# Autodesk Inventor assembly: gasienica_zlozenie
(part 2 of 2)
- [Mate]: tuleja_TUF106040:70 ↔ M6_40_shaft:7
- [Flush] (7 mm): ramie_1_wahacza:7 ↔ M6_40_shaft:7
- [Mate]: tuleja_TUF106040:73 ↔ M6_40_shaft:8
- [Flush] (7 mm): ramie_2_wahacza:8 ↔ M6_40_shaft:8
- [Mate]: M6_nut_5mm:89 ↔ M6_40_shaft:7
- [Mate]: ramie_1_wahacza:7 ↔ M6_nut_5mm:89
- [Mate]: M6_40_shaft:7 ↔ M6_nut_5mm:90
- [Mate]: ramie_1_wahacza:8 ↔ M6_nut_5mm:90
- [Mate]: M6_40_shaft:8 ↔ M6_nut_5mm:91
- [Mate]: ramie_2_wahacza:7 ↔ M6_nut_5mm:91
- [Mate]: M6_40_shaft:8 ↔ M6_nut_5mm:92
- [Mate]: ramie_2_wahacza:8 ↔ M6_nut_5mm:92
- [Mate]: M6_40_shaft:7 ↔ tuleja_M6_M10_7:10
- [Mate]: M6_40_shaft:8 ↔ tuleja_M6_M10_7:11
- [Mate]: M6_1,25_pad:25 ↔ M6_1,25_pad:26
- [Mate]: M6_1,25_pad:25 ↔ M6_1,25_pad:26
- [Mate]: M6_40_shaft:7 ↔ M6_1,25_pad:25
- [Mate]: M6_1,25_pad:27 ↔ M6_1,25_pad:28
- [Mate]: M6_1,25_pad:27 ↔ M6_1,25_pad:28
- [Mate]: M6_40_shaft:7 ↔ M6_1,25_pad:27
- [Mate]: tuleja_TUF106040:70 ↔ M6_1,25_pad:27
- [Mate]: M6_1,25_pad:29 ↔ M6_1,25_pad:30
- [Mate]: M6_1,25_pad:29 ↔ M6_1,25_pad:30
- [Mate]: M6_40_shaft:8 ↔ M6_1,25_pad:29
- [Mate]: M6_1,25_pad:31 ↔ M6_1,25_pad:32
- [Mate]: M6_1,25_pad:31 ↔ M6_1,25_pad:32
- [Mate]: M6_40_shaft:8 ↔ M6_1,25_pad:31
- [Mate]: tuleja_TUF106040:73 ↔ M6_1,25_pad:31
- [Mate]: M5_70_shaft:10 ↔ M6_70_shaft:19
- [Flush]: M5_70_shaft:10 ↔ M6_70_shaft:20
- [Mate]: M6_70_shaft:20 ↔ M6_nut_5mm:93
- [Mate]: M6_70_shaft:20 ↔ M6_nut_5mm:94
- [Mate] (60 mm): M6_nut_5mm:93 ↔ M6_nut_5mm:94
- [Flush]: M5_nut_5mm:64 ↔ M6_nut_5mm:94
- [Mate] (60 mm): M6_nut_5mm:95 ↔ M6_nut_5mm:96
- [Mate]: M6_nut_5mm:95 ↔ M6_nut_5mm:96
- [Mate]: M6_70_shaft:19 ↔ M6_nut_5mm:95
- [Flush]: M5_nut_5mm:64 ↔ M6_nut_5mm:96
- [Mate]: ramie_1_wahacza:7 ↔ M5_shaft:7
- [Flush] (7 mm): ramie_1_wahacza:7 ↔ M5_shaft:7
- [Mate]: ramie_1_wahacza:7 ↔ M5_shaft:8
- [Flush] (7 mm): ramie_1_wahacza:7 ↔ M5_shaft:8
- [Mate]: M5_shaft:8 ↔ M5_nut_5mm:66
- [Mate]: ramie_1_wahacza:7 ↔ M5_nut_5mm:66
- [Mate]: M5_shaft:7 ↔ M5_nut_5mm:67
- [Mate]: ramie_1_wahacza:7 ↔ M5_nut_5mm:67
- [Mate]: M5_shaft:7 ↔ M5_nut_5mm:68
- [Mate]: ramie_1_wahacza:8 ↔ M5_nut_5mm:68
- [Mate]: M5_shaft:8 ↔ M5_nut_5mm:69
- [Mate]: ramie_1_wahacza:8 ↔ M5_nut_5mm:69
- [Mate]: M5_shaft:7 ↔ tuleja_M5_M9_4,5:13
- [Mate]: ramie_1_wahacza:8 ↔ tuleja_M5_M9_4,5:13
- [Mate]: M5_shaft:7 ↔ tuleja_M5_M9_4,5:14
- [Mate]: ramie_1_wahacza:7 ↔ tuleja_M5_M9_4,5:14
- [Mate]: M5_shaft:8 ↔ tuleja_M5_M9_4,5:15
- [Mate]: ramie_1_wahacza:8 ↔ tuleja_M5_M9_4,5:15
- [Mate]: M5_shaft:8 ↔ tuleja_M5_M9_4,5:16
- [Mate]: ramie_1_wahacza:7 ↔ tuleja_M5_M9_4,5:16
- [Mate]: M6_40_shaft:8 ↔ glowny_wahacz_zewn:7
- [Mate]: tuleja_M6_M10_7:11 ↔ glowny_wahacz_zewn:7
- [Mate]: M6_40_shaft:7 ↔ glowny_wahacz_zewn:7
- [Mate]: M6_40_shaft:8 ↔ glowny_wahacz_zewn:8
- [Mate]: M6_40_shaft:7 ↔ glowny_wahacz_zewn:8
- [Mate]: tuleja_TUF106040:72 ↔ M6_40_shaft:7
- [Mate]: M6_1,25_pad:28 ↔ glowny_wahacz_zewn:8
- [Mate]: M6_1,25_pad:32 ↔ glowny_wahacz_zewn:8
- [Mate]: tuleja_M6_M10_7:10 ↔ glowny_wahacz_zewn:7
- [Mate]: M6_1,25_pad:25 ↔ glowny_wahacz_zewn:7
- [Mate]: tuleja_TUF106040:72 ↔ M6_1,25_pad:26
- [Mate]: M6_1,25_pad:29 ↔ glowny_wahacz_zewn:7
- [Mate]: tuleja_TUF106040:67 ↔ M6_1,25_pad:30
- [Mate]: tuleja_TUF106040:71 ↔ ramie_1_wahacza:8
- [Mate]: tuleja_TUF106040:69 ↔ M6_70_shaft:20
- [Mate]: ramie_1_wahacza:7 ↔ tuleja_TUF106040:69
- [Mate]: ramie_1_wahacza:7 ↔ tuleja_TUF106040:69
- [Mate]: tuleja_TUF106040:68 ↔ M6_70_shaft:19
- [Mate]: ramie_2_wahacza:7 ↔ tuleja_TUF106040:68
- [Mate]: ramie_2_wahacza:7 ↔ tuleja_TUF106040:68
- [Mate]: tuleja_TUF106040:74 ↔ M6_70_shaft:19
- [Mate]: ramie_2_wahacza:8 ↔ tuleja_TUF106040:74
- [Mate]: ramie_2_wahacza:8 ↔ tuleja_TUF106040:74
- [Mate]: ramie_1_wahacza:8 ↔ M5_shaft:8
- [Mate]: M6_70_shaft:19 ↔ M6_nut_5mm:97
- [Mate] (5 mm): M6_nut_5mm:96 ↔ M6_nut_5mm:97
- [Mate]: M6_70_shaft:19 ↔ M6_nut_5mm:98
- [Mate] (5 mm): M6_nut_5mm:95 ↔ M6_nut_5mm:98
- [Mate]: M6_70_shaft:20 ↔ M6_nut_5mm:99
- [Mate] (5 mm): M6_nut_5mm:93 ↔ M6_nut_5mm:99
- [Mate]: M6_70_shaft:20 ↔ M6_nut_5mm:100
- [Mate] (5 mm): M6_nut_5mm:94 ↔ M6_nut_5mm:100
- [Mate]: M6_70_shaft:20 ↔ tuleja_M6_M10_6:13
- [Mate]: tuleja_M6_M10_6:13 ↔ M6_nut_5mm:99
- [Mate]: M6_70_shaft:19 ↔ tuleja_M6_M10_6:14
- [Mate]: tuleja_TUF106040:74 ↔ tuleja_M6_M10_6:14
- [Mate]: M6_70_shaft:19 ↔ tuleja_M6_M10_6:15
- [Mate]: tuleja_TUF106040:68 ↔ tuleja_M6_M10_6:15
- [Mate]: M6_70_shaft:20 ↔ tuleja_M6_M10_6:16
- [Mate]: tuleja_TUF106040:71 ↔ tuleja_M6_M10_6:16
- [Mate]: M5_70_shaft:10 ↔ M5_nut_5mm:70
- [Mate] (5 mm): M5_nut_5mm:64 ↔ M5_nut_5mm:70
- [Mate]: M5_70_shaft:10 ↔ M5_nut_5mm:71
- [Mate] (5 mm): M5_nut_5mm:65 ↔ M5_nut_5mm:71
- [Mate]: M5_70_shaft:10 ↔ tuleja_M5_M9_17.5:8
- [Mate]: M5_nut_5mm:71 ↔ tuleja_M5_M9_17.5:8
- [Mate]: M5_70_shaft:10 ↔ tuleja_M5_M9_17.5:7
- [Mate]: Korpus:10 ↔ tuleja_M5_M9_17.5:7
- Zestawiające:1632 [Mate]: plyta_boczna:1 ↔ M6_70_shaft:16
- Zestawiające:1633 [Mate]: plyta_boczna:1 ↔ M6_nut_5mm:75
- Zestawiające:1636 [Mate]: plyta_boczna:2 ↔ M6_70_shaft:15
- Zestawiające:1637 [Mate]: plyta_boczna:2 ↔ tuleja_M5_M9_17.5:3
- Kątowe:40 [Angle] (90 deg): ramie_1_wahacza:4 ↔ glowny_wahacz_zewn:3
- Zestawiające:1638 [Mate]: plyta_boczna:2 ↔ M5_nut_5mm:65
- Zestawiające:1639 [Mate]: plyta_boczna:2 ↔ M6_70_shaft:20
- Zestawiające:1640 [Mate]: plyta_boczna:2 ↔ M6_70_shaft:19
- Zestawiające:1641 [Mate]: plyta_boczna:2 ↔ tuleja_M5_M9_17.5:7
- Kątowe:41 [Angle] (90 deg): ramie_1_wahacza:7 ↔ glowny_wahacz_zewn:8
- [Mate]: ramie_2_wahacza:9 ↔ tuleja_TUF106040:75
- [Mate]: ramie_2_wahacza:9 ↔ tuleja_TUF106040:75
- [Angle] (0 deg): ramie_2_wahacza:9 ↔ tuleja_TUF106040:75
- [Mate]: ramie_1_wahacza:9 ↔ tuleja_TUF106040:78
- [Mate]: ramie_1_wahacza:9 ↔ tuleja_TUF106040:78
- [Angle] (0 deg): ramie_1_wahacza:9 ↔ tuleja_TUF106040:78
- [Mate]: ramie_2_wahacza:10 ↔ tuleja_TUF106040:81
- [Mate]: ramie_2_wahacza:10 ↔ tuleja_TUF106040:81
- [Angle] (0 deg): ramie_2_wahacza:10 ↔ tuleja_TUF106040:81
- [Mate]: Korpus:11 ↔ Tlok:11
- [Angle] (0 deg): Korpus:11 ↔ Tlok:11
- [Mate]: Korpus:11 ↔ Nakretka:11
- [Mate] (5 mm): Korpus:11 ↔ Nakretka:11
- [CylindricalJoint]: Korpus:11 ↔ Tlok:11
- [Mate]: Korpus:11 ↔ M5_70_shaft:11
- [Flush] (-32.5 mm): Korpus:11 ↔ M5_70_shaft:11
- [Mate]: M5_nut_5mm:72 ↔ M5_70_shaft:11
- [Mate]: M5_70_shaft:11 ↔ M5_nut_5mm:73
- [Mate] (60 mm): M5_nut_5mm:72 ↔ M5_nut_5mm:73
- [Mate] (27.5 mm): Korpus:11 ↔ M5_nut_5mm:72
- [Mate]: tuleja_TUF106040:80 ↔ ramie_1_wahacza:10
- [Mate]: tuleja_TUF106040:79 ↔ ramie_1_wahacza:10
- [Mate]: tuleja_TUF106040:80 ↔ ramie_1_wahacza:10
- [Mate]: tuleja_TUF106040:75 ↔ tuleja_TUF106040:81
- [Mate]: wspornik_amortyzatora:21 ↔ wspornik_amortyzatora:22
- [Mate]: wspornik_amortyzatora:21 ↔ wspornik_amortyzatora:22
- [Mate] (5 mm): wspornik_amortyzatora:21 ↔ wspornik_amortyzatora:22
- [Mate]: M3_16_shaft:11 ↔ wspornik_amortyzatora:22
- [Flush] (-2.5 mm): M3_16_shaft:11 ↔ wspornik_amortyzatora:21
- [Mate]: M3_16_shaft:11 ↔ M3_nut_2,5mm:21
- [Mate]: M3_nut_2,5mm:21 ↔ wspornik_amortyzatora:21
- [Mate]: M3_16_shaft:11 ↔ M3_nut_2,5mm:22
- [Mate]: M3_nut_2,5mm:22 ↔ wspornik_amortyzatora:22
- [Mate]: Tlok:11 ↔ M3_16_shaft:11
- [Mate]: Tlok:11 ↔ wspornik_amortyzatora:22
- [Mate]: ramie_1_wahacza:9 ↔ wspornik_amortyzatora:21
- [Mate]: ramie_1_wahacza:9 ↔ wspornik_amortyzatora:21
- [Mate] (4.5 mm): ramie_1_wahacza:9 ↔ wspornik_amortyzatora:21
- [Mate]: tuleja_TUF106040:78 ↔ M6_40_shaft:9
- [Flush] (7 mm): ramie_1_wahacza:9 ↔ M6_40_shaft:9
- [Mate]: tuleja_TUF106040:81 ↔ M6_40_shaft:10
- [Flush] (7 mm): ramie_2_wahacza:10 ↔ M6_40_shaft:10
- [Mate]: M6_nut_5mm:101 ↔ M6_40_shaft:9
- [Mate]: ramie_1_wahacza:9 ↔ M6_nut_5mm:101
- [Mate]: M6_40_shaft:9 ↔ M6_nut_5mm:102
- [Mate]: ramie_1_wahacza:10 ↔ M6_nut_5mm:102
- [Mate]: M6_40_shaft:10 ↔ M6_nut_5mm:103
- [Mate]: ramie_2_wahacza:9 ↔ M6_nut_5mm:103
- [Mate]: M6_40_shaft:10 ↔ M6_nut_5mm:104
- [Mate]: ramie_2_wahacza:10 ↔ M6_nut_5mm:104
- [Mate]: M6_40_shaft:9 ↔ tuleja_M6_M10_7:13
- [Mate]: M6_40_shaft:10 ↔ tuleja_M6_M10_7:14
- [Mate]: M6_1,25_pad:33 ↔ M6_1,25_pad:34
- [Mate]: M6_1,25_pad:33 ↔ M6_1,25_pad:34
- [Mate]: M6_40_shaft:9 ↔ M6_1,25_pad:33
- [Mate]: M6_1,25_pad:35 ↔ M6_1,25_pad:36
- [Mate]: M6_1,25_pad:35 ↔ M6_1,25_pad:36
- [Mate]: M6_40_shaft:9 ↔ M6_1,25_pad:35
- [Mate]: tuleja_TUF106040:78 ↔ M6_1,25_pad:35
- [Mate]: M6_1,25_pad:37 ↔ M6_1,25_pad:38
- [Mate]: M6_1,25_pad:37 ↔ M6_1,25_pad:38
- [Mate]: M6_40_shaft:10 ↔ M6_1,25_pad:37
- [Mate]: M6_1,25_pad:39 ↔ M6_1,25_pad:40
- [Mate]: M6_1,25_pad:39 ↔ M6_1,25_pad:40
- [Mate]: M6_40_shaft:10 ↔ M6_1,25_pad:39
- [Mate]: tuleja_TUF106040:81 ↔ M6_1,25_pad:39
- [Mate]: M5_70_shaft:11 ↔ M6_70_shaft:21
- [Flush]: M5_70_shaft:11 ↔ M6_70_shaft:22
- [Mate]: M6_70_shaft:22 ↔ M6_nut_5mm:105
- [Mate]: M6_70_shaft:22 ↔ M6_nut_5mm:106
- [Mate] (60 mm): M6_nut_5mm:105 ↔ M6_nut_5mm:106
- [Flush]: M5_nut_5mm:72 ↔ M6_nut_5mm:106
- [Mate] (60 mm): M6_nut_5mm:107 ↔ M6_nut_5mm:108
- [Mate]: M6_nut_5mm:107 ↔ M6_nut_5mm:108
- [Mate]: M6_70_shaft:21 ↔ M6_nut_5mm:107
- [Flush]: M5_nut_5mm:72 ↔ M6_nut_5mm:108
- [Mate]: ramie_1_wahacza:9 ↔ M5_shaft:9
- [Flush] (7 mm): ramie_1_wahacza:9 ↔ M5_shaft:9
- [Mate]: ramie_1_wahacza:9 ↔ M5_shaft:10
- [Flush] (7 mm): ramie_1_wahacza:9 ↔ M5_shaft:10
- [Mate]: M5_shaft:10 ↔ M5_nut_5mm:74
- [Mate]: ramie_1_wahacza:9 ↔ M5_nut_5mm:74
- [Mate]: M5_shaft:9 ↔ M5_nut_5mm:75
- [Mate]: ramie_1_wahacza:9 ↔ M5_nut_5mm:75
- [Mate]: M5_shaft:9 ↔ M5_nut_5mm:76
- [Mate]: ramie_1_wahacza:10 ↔ M5_nut_5mm:76
- [Mate]: M5_shaft:10 ↔ M5_nut_5mm:77
- [Mate]: ramie_1_wahacza:10 ↔ M5_nut_5mm:77
- [Mate]: M5_shaft:9 ↔ tuleja_M5_M9_4,5:17
- [Mate]: ramie_1_wahacza:10 ↔ tuleja_M5_M9_4,5:17
- [Mate]: M5_shaft:9 ↔ tuleja_M5_M9_4,5:18
- [Mate]: ramie_1_wahacza:9 ↔ tuleja_M5_M9_4,5:18
- [Mate]: M5_shaft:10 ↔ tuleja_M5_M9_4,5:19
- [Mate]: ramie_1_wahacza:10 ↔ tuleja_M5_M9_4,5:19
- [Mate]: M5_shaft:10 ↔ tuleja_M5_M9_4,5:20
- [Mate]: ramie_1_wahacza:9 ↔ tuleja_M5_M9_4,5:20
- [Mate]: M6_40_shaft:10 ↔ glowny_wahacz_zewn:9
- [Mate]: tuleja_M6_M10_7:14 ↔ glowny_wahacz_zewn:9
- [Mate]: M6_40_shaft:9 ↔ glowny_wahacz_zewn:9
- [Mate]: M6_40_shaft:10 ↔ glowny_wahacz_zewn:10
- [Mate]: M6_40_shaft:9 ↔ glowny_wahacz_zewn:10
- [Mate]: tuleja_TUF106040:80 ↔ M6_40_shaft:9
- [Mate]: M6_1,25_pad:36 ↔ glowny_wahacz_zewn:10
- [Mate]: M6_1,25_pad:40 ↔ glowny_wahacz_zewn:10
- [Mate]: tuleja_M6_M10_7:13 ↔ glowny_wahacz_zewn:9
- [Mate]: M6_1,25_pad:33 ↔ glowny_wahacz_zewn:9
- [Mate]: tuleja_TUF106040:80 ↔ M6_1,25_pad:34
- [Mate]: M6_1,25_pad:37 ↔ glowny_wahacz_zewn:9
- [Mate]: tuleja_TUF106040:75 ↔ M6_1,25_pad:38
- [Mate]: tuleja_TUF106040:79 ↔ ramie_1_wahacza:10
- [Mate]: tuleja_TUF106040:77 ↔ M6_70_shaft:22
- [Mate]: ramie_1_wahacza:9 ↔ tuleja_TUF106040:77
- [Mate]: ramie_1_wahacza:9 ↔ tuleja_TUF106040:77
- [Mate]: tuleja_TUF106040:76 ↔ M6_70_shaft:21
- [Mate]: ramie_2_wahacza:9 ↔ tuleja_TUF106040:76
- [Mate]: ramie_2_wahacza:9 ↔ tuleja_TUF106040:76
- [Mate]: tuleja_TUF106040:82 ↔ M6_70_shaft:21
- [Mate]: ramie_2_wahacza:10 ↔ tuleja_TUF106040:82
- [Mate]: ramie_2_wahacza:10 ↔ tuleja_TUF106040:82
- [Mate]: independent_wheel_pair:5 ↔ tuleja_M6_M10_7:15
- [Mate]: glowny_wahacz_zewn:10 ↔ independent_wheel_pair:5
- [Mate]: glowny_wahacz_zewn:10 ↔ independent_wheel_pair:5
- [Mate]: glowny_wahacz_zewn:10 ↔ tuleja_M6_M10_7:15
- [Mate]: ramie_1_wahacza:10 ↔ M5_shaft:10
- [Mate]: M6_70_shaft:21 ↔ M6_nut_5mm:109
- [Mate] (5 mm): M6_nut_5mm:108 ↔ M6_nut_5mm:109
- [Mate]: M6_70_shaft:21 ↔ M6_nut_5mm:110
- [Mate] (5 mm): M6_nut_5mm:107 ↔ M6_nut_5mm:110
- [Mate]: M6_70_shaft:22 ↔ M6_nut_5mm:111
- [Mate] (5 mm): M6_nut_5mm:105 ↔ M6_nut_5mm:111
- [Mate]: M6_70_shaft:22 ↔ M6_nut_5mm:112
- [Mate] (5 mm): M6_nut_5mm:106 ↔ M6_nut_5mm:112
- [Mate]: M6_70_shaft:22 ↔ tuleja_M6_M10_6:17
- [Mate]: tuleja_M6_M10_6:17 ↔ M6_nut_5mm:111
- [Mate]: M6_70_shaft:21 ↔ tuleja_M6_M10_6:18
- [Mate]: tuleja_TUF106040:82 ↔ tuleja_M6_M10_6:18
- [Mate]: M6_70_shaft:21 ↔ tuleja_M6_M10_6:19
- [Mate]: tuleja_TUF106040:76 ↔ tuleja_M6_M10_6:19
- [Mate]: M6_70_shaft:22 ↔ tuleja_M6_M10_6:20
- [Mate]: tuleja_TUF106040:79 ↔ tuleja_M6_M10_6:20
- [Mate]: M5_70_shaft:11 ↔ M5_nut_5mm:78
- [Mate] (5 mm): M5_nut_5mm:72 ↔ M5_nut_5mm:78
- [Mate]: M5_70_shaft:11 ↔ M5_nut_5mm:79
- [Mate] (5 mm): M5_nut_5mm:73 ↔ M5_nut_5mm:79
- [Mate]: M5_70_shaft:11 ↔ tuleja_M5_M9_17.5:10
- [Mate]: M5_nut_5mm:79 ↔ tuleja_M5_M9_17.5:10
- [Mate]: M5_70_shaft:11 ↔ tuleja_M5_M9_17.5:9
- [Mate]: Korpus:11 ↔ tuleja_M5_M9_17.5:9
- [Mate]: glowny_wahacz_zewn:9 ↔ independent_wheel_pair:5
- Zestawiające:1777 [Mate]: plyta_boczna:2 ↔ M6_nut_5mm:107
- Zestawiające:1778 [Mate]: plyta_boczna:2 ↔ M6_70_shaft:22
- Zestawiające:1779 [Mate]: plyta_boczna:2 ↔ M6_70_shaft:21
- Zestawiające:1780 [Mate]: plyta_boczna:2 ↔ tuleja_M5_M9_17.5:10
- Kątowe:47 [Angle] (90 deg): ramie_1_wahacza:9 ↔ glowny_wahacz_zewn:10
- Zestawiające:1781 [Mate]: glowny_wahacz_zewn:8 ↔ komplet_kol_V4:1
- Zestawiające:1782 [Mate]: glowny_wahacz_zewn:8 ↔ komplet_kol_V4:1
- Zestawiające:1784 [Mate]: glowny_wahacz_zewn:7 ↔ komplet_kol_V4:1
- [Mate]: M6_25_shaft:2 ↔ M6_nut_5mm:116
- [Mate]: M6_nut_5mm:115 ↔ M6_25_shaft:2
- [Flush] (-1 mm): M6_nut_5mm:115 ↔ M6_25_shaft:2
- [Flush] (1 mm): M6_25_shaft:2 ↔ M6_nut_5mm:116
- Zestawiające:1788 [Mate]: komplet_kol_V4:1 ↔ M6_25_shaft:2
- Zestawiające:1789 [Mate]: glowny_wahacz_zewn:8 ↔ M6_nut_5mm:115
- [Mate]: M6_25_shaft:3 ↔ M6_nut_5mm:118
- [Mate]: M6_nut_5mm:117 ↔ M6_25_shaft:3
- [Flush] (-1 mm): M6_nut_5mm:117 ↔ M6_25_shaft:3
- [Flush] (1 mm): M6_25_shaft:3 ↔ M6_nut_5mm:118
- [Mate]: komplet_kol_V4:2 ↔ M6_25_shaft:3
- Zestawiające:1793 [Mate] (7 mm): glowny_wahacz_zewn:3 ↔ glowny_wahacz_zewn:4
- Zestawiające:1794 [Mate]: glowny_wahacz_zewn:3 ↔ M6_25_shaft:3
- Zestawiające:1795 [Mate]: glowny_wahacz_zewn:3 ↔ komplet_kol_V4:2
- Kątowe:48 [Angle] (0 deg): komplet_kol_V4:1 ↔ komplet_kol_V4:2
- Kątowe:49 [Angle] (0 deg): plyta_boczna:1 ↔ komplet_kol_V4:2
- Zestawiające:1796 [Mate]: M5_60_shaft:2 ↔ tuleja_M5_M9_13:1
- Zestawiające:1797 [Mate]: M5_60_shaft:2 ↔ tuleja_M5_M9_18:1
- [Mate]: single_wheel_dummie:1 ↔ tuleja_M5_M10_15:1
- Zestawiające:1799 [Mate]: single_wheel_dummie:1 ↔ tuleja_M5_M10_15:1
- Zestawiające:1800 [Mate]: single_wheel_dummie:2 ↔ tuleja_M5_M10_15:1
- Zestawiające:1801 [Mate]: single_wheel_dummie:2 ↔ tuleja_M5_M10_15:1
- Zestawiające:1802 [Mate]: M6_70_shaft:11 ↔ single_wheel_dummie:2
- Zestawiające:1803 [Mate]: M6_70_shaft:11 ↔ tuleja_M6_M10_7,5:1
- Zestawiające:1804 [Mate]: ramie_napinacza:2 ↔ tuleja_M6_M10_7,5:1
- Zestawiające:1805 [Mate]: single_wheel_dummie:2 ↔ tuleja_M6_M10_7,5:1
- Zestawiające:1806 [Mate]: M6_70_shaft:11 ↔ tuleja_M6_M10_7,5:2
- Zestawiające:1807 [Mate]: ramie_napinacza:1 ↔ tuleja_M6_M10_7,5:2
## Named parameters: d25_d17_d47_d24 = 0 mm, d26_d18_d48_d25 = 0 mm, d27_d19_d15 = 0 mm, d28_d20_d16 = 5 mm, d102_d31 = 0 mm, d103_d32 = 7 mm, d104_d33 = 0 mm, d105_d34 = 0 mm, d705_d35 = 0 mm, d706_d36 = 31 mm, d707_d37 = 0 mm, d109_d23 = 0 mm, d110_d24 = 0 mm, d111_d25 = 0 mm, d112_d26 = 0 mm, d113_d27 = 7 mm, d114_d28 = 0 mm, d115_d30 = 0 mm, d715_d116 = 0 mm, d716_d117 = 0 mm, d717_d118 = 0 mm, d718_d119 = 0 mm, susp_angle = 90 deg, tlok_scisniety = -13 mm, tlok_wyprostowany = 1 mm, d1532_d239 = 0 mm, d1533_d174 = 0 mm, d1534_d175 = 0 mm, d1535_d176 = 60 mm, d1545_d86_d0 = 0 mm, d1546_d87_d1 = 0 deg, d1547_d88_d3 = 0 mm, d1548_d89_d4 = 5 mm, d1549_d90_d5 = 0 deg, d1550_d108 = 0 mm, d1551_d109 = -30 mm, d1552_d110 = 0 mm, d1553_d111 = 0 mm, d1554_d112 = 60 mm, d1555_d113 = 30 mm, d1587_d202 = 0 mm, d1588_d203 = 0 mm, d1589_d204 = 0 mm, d1590_d205 = 0 mm, d1591_d120 = 0 mm, d1592_d121 = 0 mm, d1593_d122 = 5 mm, d1594_d123 = 0 mm, d1595_d124 = -2.5 mm, d1596_d125 = 0 mm, d1597_d126 = 0 mm, d1598_d127 = 0 mm, d1599_d128 = 0 mm, d1600_d129 = 0 mm, d1601_d130 = 0 mm, d1602_d83_d6 = 0 mm, d1603_d84_d7 = -13 mm, d1604_d85_d8 = -13 mm, d1684_d208 = 0 mm, d1685_d209 = 0 mm, d158_d154 = 0 mm, d159_d155 = 0 mm, d162_d154 = 0 mm, d163_d155 = 0 mm, d166_d154 = 0 mm, d167_d155 = 0 mm, d178_d176 = 60 mm, d41_d4 = 0 deg, d43_d0 = 0 mm, d44_d1 = 0 mm, d83_d6 = 0 mm, d84_d7 = -5.94197 mm, d85_d8 = -13 mm, d86_d0 = 0 mm, d87_d1 = 0 deg, d88_d3 = 0 mm, d89_d4 = 5 mm, d90_d5 = 0 deg, d1784_d333 = 5 mm, d1785_d334 = 0 mm, d1786_d335 = 5 mm, d1787_d336 = 0 mm, d1788_d337 = 0 mm, d1789_d338 = 0 mm, d1790_d339 = 0 mm, d1792_d321 = 5 mm, d1793_d322 = 0 mm, d1794_d323 = 5 mm, d1795_d324 = 0 mm, d1796_d325 = 0 mm, d1797_d326 = 0 mm, d1798_d327 = 0 mm, d1799_d328 = 0 mm, d1800_d329 = 0 mm, d1801_d330 = 0 mm, d1802_d331 = 0 mm, d1803_d332 = 0 mm, d1804_d0 = 0 mm, d1805_d1 = 0 mm, d1806_d4 = 0 deg, d1807_d9 = 0 mm, d1808_d315 = 0 mm, d1809_d316 = 0 mm, d1810_d317 = 5 mm, d1811_d318 = 0 mm, d1812_d319 = 5 mm, d1813_d320 = 0 mm, d1814_d233 = 0 mm, d1815_d234 = 0 mm, d1816_d235 = 0 mm, d1817_d236 = 0 mm, d1818_d237 = 0 mm, d1819_d238 = 0 mm, d1820_d239 = 0 mm, d1821_d240 = 0 mm, d1822_d241 = 0 mm, d1823_d242 = 0 mm, d1824_d243 = 0 mm, d1825_d244 = 0 mm, d1826_d245 = 0 mm, d1827_d246 = 0 mm, d1828_d247 = 0 mm, d1833_d195 = 0 mm, d1834_d196 = 0 mm, d1835_d197 = 0 mm, d1836_d198 = 0 mm, d1837_d199 = 0 mm, d1838_d200 = 0 mm, d1839_d201 = 0 mm, d1840_d206 = 0 mm, d1841_d207 = 0 mm, d1842_d208 = 0 mm, d1843_d209 = 0 mm, d1844_d210 = 0 mm, d1845_d211 = 0 mm, d1846_d212 = 0 mm, d1847_d213 = 0 mm, d1848_d216 = 0 mm, d1849_d217 = 0 mm, d1850_d218 = 0 mm, d1851_d221 = 0 mm, d1852_d222 = 0 mm, d1853_d225 = 0 mm, d1854_d231 = 0 mm, d1855_d232 = 0 mm, d1856_d154 = 0 mm, d1857_d155 = 0 mm, d1858_d156 = 0 mm, d1859_d158_d154 = 0 mm, d1860_d159_d155 = 0 mm, d1861_d160 = 0 mm, d1862_d161 = 0 mm, d1863_d162_d154 = 0 mm, d1864_d163_d155 = 0 mm, d1865_d164 = 0 mm, d1866_d166_d154 = 0 mm, d1867_d167_d155 = 0 mm, d1868_d168 = 0 mm, d1869_d169 = 0 mm, d1870_d172 = 0 mm, d1871_d173 = 0 mm, d1872_d174 = 0 mm, d1873_d175 = 0 mm, d1874_d176 = 60 mm, d1875_d177 = 0 mm, d1876_d178_d176 = 60 mm, d1877_d179 = 0 mm, d1878_d180 = 0 mm, d1879_d181 = 0 mm, d1880_d190 = 0 mm, d1881_d191 = 7 mm, d1882_d192 = 0 mm, d1883_d193 = 7 mm, d1884_d194 = 0 mm, d1885_d119 = 0 mm, d1886_d120 = 0 mm, d1887_d121 = 0 mm, d1888_d122 = 5 mm, d1889_d123 = 0 mm, d1890_d124 = -2.5 mm, d1891_d125 = 0 mm, d1892_d126 = 0 mm, d1893_d127 = 0 mm, d1894_d128 = 0 mm, d1895_d129 = 0 mm, d1896_d130 = 0 mm, d1897_d135 = 0 mm, d1898_d136 = 0 mm, d1899_d137 = 4.5 mm, d1900_d138 = 0 mm, d1901_d139 = 7 mm, d1902_d140 = 0 mm, d1903_d141 = 7 mm, d1904_d142 = 0 mm, d1905_d143 = 0 mm, d1906_d144 = 0 mm, d1907_d145 = 0 mm, d1908_d146 = 0 mm, d1909_d147 = 0 mm, d1910_d148 = 0 mm, d1911_d149 = 0 mm, d1912_d150 = 0 mm, d1913_d152 = 0 mm, d1914_d10 = 0 mm, d1915_d11 = 0 deg, d1916_d41_d4 = 0 deg, d1917_d43_d0 = 0 mm, d1918_d44_d1 = 0 mm, d1919_d83_d6 = 0 mm, d1920_d84_d7 = -5.942 mm, d1921_d85_d8 = -13 mm, d1922_d86_d0 = 0 mm, d1923_d87_d1 = 0 deg, d1924_d88_d3 = 0 mm, d1925_d89_d4 = 5 mm, d1926_d90_d5 = 0 deg, d1927_d108 = 0 mm, d1928_d109 = -32.5 mm, d1929_d110 = 0 mm, d1930_d111 = 0 mm, d1931_d112 = 60 mm, d1932_d113 = 27.5 mm, d1933_d114 = 0 mm, d1934_d115 = 0 mm, d1935_d116 = 0 mm, d2088_d333 = 5 mm, d2089_d334 = 0 mm, d2090_d335 = 5 mm, d2091_d336 = 0 mm, d2092_d337 = 0 mm, d2093_d338 = 0 mm, d2094_d339 = 0 mm, d2096_d321 = 5 mm, d2097_d322 = 0 mm, d2098_d323 = 5 mm, d2099_d324 = 0 mm, d2100_d325 = 0 mm, d2101_d326 = 0 mm, d2102_d327 = 0 mm, d2103_d328 = 0 mm, d2104_d329 = 0 mm, d2105_d330 = 0 mm, d2106_d331 = 0 mm, d2107_d332 = 0 mm, d2108_d0 = 0 mm, d2109_d1 = 0 mm, d2110_d4 = 0 deg, d2111_d9 = 0 mm, d2112_d315 = 0 mm, d2113_d316 = 0 mm, d2114_d317 = 5 mm, d2115_d318 = 0 mm, d2116_d319 = 5 mm, d2117_d320 = 0 mm, d2118_d233 = 0 mm, d2119_d234 = 0 mm, d2120_d235 = 0 mm, d2121_d236 = 0 mm, d2122_d237 = 0 mm, d2123_d238 = 0 mm, d2124_d239 = 0 mm, d2125_d240 = 0 mm, d2126_d241 = 0 mm, d2127_d242 = 0 mm, d2128_d243 = 0 mm, d2129_d244 = 0 mm, d2130_d245 = 0 mm, d2131_d246 = 0 mm, d2132_d247 = 0 mm, d2137_d195 = 0 mm, d2138_d196 = 0 mm, d2139_d197 = 0 mm, d2140_d198 = 0 mm, d2141_d199 = 0 mm, d2142_d200 = 0 mm, d2143_d201 = 0 mm, d2144_d206 = 0 mm, d2145_d207 = 0 mm, d2146_d208 = 0 mm, d2147_d209 = 0 mm, d2148_d210 = 0 mm, d2149_d211 = 0 mm, d2150_d212 = 0 mm, d2151_d213 = 0 mm, d2152_d216 = 0 mm, d2153_d217 = 0 mm, d2154_d218 = 0 mm, d2155_d221 = 0 mm, d2156_d222 = 0 mm, d2157_d225 = 0 mm, d2158_d231 = 0 mm, d2159_d232 = 0 mm, d2160_d154 = 0 mm, d2161_d155 = 0 mm, d2162_d156 = 0 mm, d2163_d158_d154 = 0 mm, d2164_d159_d155 = 0 mm, d2165_d160 = 0 mm, d2166_d161 = 0 mm, d2167_d162_d154 = 0 mm, d2168_d163_d155 = 0 mm, d2169_d164 = 0 mm, d2170_d166_d154 = 0 mm, d2171_d167_d155 = 0 mm, d2172_d168 = 0 mm, d2173_d169 = 0 mm, d2174_d172 = 0 mm, d2175_d173 = 0 mm, d2176_d174 = 0 mm, d2177_d175 = 0 mm, d2178_d176 = 60 mm, d2179_d177 = 0 mm, d2180_d178_d176 = 60 mm, d2181_d179 = 0 mm, d2182_d180 = 0 mm, d2183_d181 = 0 mm, d2184_d190 = 0 mm, d2185_d191 = 7 mm, d2186_d192 = 0 mm, d2187_d193 = 7 mm, d2188_d194 = 0 mm, d2189_d119 = 0 mm, d2190_d120 = 0 mm, d2191_d121 = 0 mm, d2192_d122 = 5 mm, d2193_d123 = 0 mm, d2194_d124 = -2.5 mm, d2195_d125 = 0 mm, d2196_d126 = 0 mm, d2197_d127 = 0 mm, d2198_d128 = 0 mm, d2199_d129 = 0 mm, d2200_d130 = 0 mm, d2201_d135 = 0 mm, d2202_d136 = 0 mm, d2203_d137 = 4.5 mm, d2204_d138 = 0 mm, d2205_d139 = 7 mm, d2206_d140 = 0 mm, d2207_d141 = 7 mm, d2208_d142 = 0 mm, d2209_d143 = 0 mm, d2210_d144 = 0 mm, d2211_d145 = 0 mm, d2212_d146 = 0 mm, d2213_d147 = 0 mm, d2214_d148 = 0 mm, d2215_d149 = 0 mm, d2216_d150 = 0 mm, d2217_d152 = 0 mm, d2218_d10 = 0 mm, d2219_d11 = 0 deg, d2220_d41_d4 = 0 deg, d2221_d43_d0 = 0 mm, d2222_d44_d1 = 0 mm, d2223_d83_d6 = 0 mm, d2224_d84_d7 = -5.942 mm, d2225_d85_d8 = -13 mm, d2226_d86_d0 = 0 mm, d2227_d87_d1 = 0 deg, d2228_d88_d3 = 0 mm, d2229_d89_d4 = 5 mm, d2230_d90_d5 = 0 deg, d2231_d108 = 0 mm, d2232_d109 = -32.5 mm, d2233_d110 = 0 mm, d2234_d111 = 0 mm, d2235_d112 = 60 mm, d2236_d113 = 27.5 mm, d2237_d114 = 0 mm, d2238_d115 = 0 mm, d2239_d116 = 0 mm, d2252_d2088_d333 = 5 mm, d2253_d2089_d334 = 0 mm, d2254_d2090_d335 = 5 mm, d2255_d2091_d336 = 0 mm, d2256_d2092_d337 = 0 mm, d2257_d2093_d338 = 0 mm, d2258_d2094_d339 = 0 mm, d2259_d2095_d340 = 0 mm, d2260_d2096_d321 = 5 mm, d2261_d2097_d322 = 0 mm, d2262_d2098_d323 = 5 mm, d2263_d2099_d324 = 0 mm, d2264_d2100_d325 = 0 mm, d2265_d2101_d326 = 0 mm, d2266_d2102_d327 = 0 mm, d2267_d2103_d328 = 0 mm, d2268_d2104_d329 = 0 mm, d2269_d2105_d330 = 0 mm, d2270_d2106_d331 = 0 mm, d2271_d2107_d332 = 0 mm, d2272_d2108_d0 = 0 mm, d2273_d2109_d1 = 0 mm, d2274_d2110_d4 = 0 deg, d2275_d2111_d9 = 0 mm, d2276_d2112_d315 = 0 mm, d2277_d2113_d316 = 0 mm, d2278_d2114_d317 = 5 mm, d2279_d2115_d318 = 0 mm, d2280_d2116_d319 = 5 mm, d2281_d2117_d320 = 0 mm, d2282_d2118_d233 = 0 mm, d2283_d2119_d234 = 0 mm, d2284_d2120_d235 = 0 mm, d2285_d2121_d236 = 0 mm, d2286_d2122_d237 = 0 mm, d2287_d2123_d238 = 0 mm, d2288_d2124_d239 = 0 mm, d2289_d2125_d240 = 0 mm, d2290_d2126_d241 = 0 mm, d2291_d2127_d242 = 0 mm, d2292_d2128_d243 = 0 mm, d2293_d2129_d244 = 0 mm, d2294_d2130_d245 = 0 mm, d2295_d2131_d246 = 0 mm, d2296_d2132_d247 = 0 mm, d2297_d2133_d1369 = 0 mm, d2298_d2134_d260 = 0 mm, d2299_d2135_d261 = 0 mm, d2300_d2136_d262 = 0 mm, d2301_d2137_d195 = 0 mm, d2302_d2138_d196 = 0 mm, d2303_d2139_d197 = 0 mm, d2304_d2140_d198 = 0 mm, d2305_d2141_d199 = 0 mm, d2306_d2142_d200 = 0 mm, d2307_d2143_d201 = 0 mm, d2308_d2144_d206 = 0 mm, d2309_d2145_d207 = 0 mm, d2310_d2146_d208 = 0 mm, d2311_d2147_d209 = 0 mm, d2312_d2148_d210 = 0 mm, d2313_d2149_d211 = 0 mm, d2314_d2150_d212 = 0 mm, d2315_d2151_d213 = 0 mm, d2316_d2152_d216 = 0 mm, d2317_d2153_d217 = 0 mm, d2318_d2154_d218 = 0 mm, d2319_d2155_d221 = 0 mm, d2320_d2156_d222 = 0 mm, d2321_d2157_d225 = 0 mm, d2322_d2158_d231 = 0 mm, d2323_d2159_d232 = 0 mm, d2324_d2160_d154 = 0 mm, d2325_d2161_d155 = 0 mm, d2326_d2162_d156 = 0 mm, d2327_d2163_d158_d154 = 0 mm, d2328_d2164_d159_d155 = 0 mm, d2329_d2165_d160 = 0 mm, d2330_d2166_d161 = 0 mm, d2331_d2167_d162_d154 = 0 mm, d2332_d2168_d163_d155 = 0 mm, d2333_d2169_d164 = 0 mm, d2334_d2170_d166_d154 = 0 mm, d2335_d2171_d167_d155 = 0 mm, d2336_d2172_d168 = 0 mm, d2337_d2173_d169 = 0 mm, d2338_d2174_d172 = 0 mm, d2339_d2175_d173 = 0 mm, d2340_d2176_d174 = 0 mm, d2341_d2177_d175 = 0 mm, d2342_d2178_d176 = 60 mm, d2343_d2179_d177 = 0 mm, d2344_d2180_d178_d176 = 60 mm, d2345_d2181_d179 = 0 mm, d2346_d2182_d180 = 0 mm, d2347_d2183_d181 = 0 mm, d2348_d2184_d190 = 0 mm, d2349_d2185_d191 = 7 mm, d2350_d2186_d192 = 0 mm, d2351_d2187_d193 = 7 mm, d2352_d2188_d194 = 0 mm, d2353_d2189_d119 = 0 mm, d2354_d2190_d120 = 0 mm, d2355_d2191_d121 = 0 mm, d2356_d2192_d122 = 5 mm, d2357_d2193_d123 = 0 mm, d2358_d2194_d124 = -2.5 mm, d2359_d2195_d125 = 0 mm, d2360_d2196_d126 = 0 mm, d2361_d2197_d127 = 0 mm, d2362_d2198_d128 = 0 mm, d2363_d2199_d129 = 0 mm, d2364_d2200_d130 = 0 mm, d2365_d2201_d135 = 0 mm, d2366_d2202_d136 = 0 mm, d2367_d2203_d137 = 4.5 mm, d2368_d2204_d138 = 0 mm, d2369_d2205_d139 = 7 mm, d2370_d2206_d140 = 0 mm, d2371_d2207_d141 = 7 mm, d2372_d2208_d142 = 0 mm, d2373_d2209_d143 = 0 mm, d2374_d2210_d144 = 0 mm, d2375_d2211_d145 = 0 mm, d2376_d2212_d146 = 0 mm, d2377_d2213_d147 = 0 mm, d2378_d2214_d148 = 0 mm, d2379_d2215_d149 = 0 mm, d2380_d2216_d150 = 0 mm, d2381_d2217_d152 = 0 mm, d2382_d2218_d10 = 0 mm, d2383_d2219_d11 = 0 deg, d2384_d2220_d41_d4 = 0 deg, d2385_d2221_d43_d0 = 0 mm, d2386_d2222_d44_d1 = 0 mm, d2387_d2223_d83_d6 = 0 mm, d2388_d2224_d84_d7 = -5.942 mm, d2389_d2225_d85_d8 = -13 mm, d2390_d2226_d86_d0 = 0 mm, d2391_d2227_d87_d1 = 0 deg, d2392_d2228_d88_d3 = 0 mm, d2393_d2229_d89_d4 = 5 mm, d2394_d2230_d90_d5 = 0 deg, d2395_d2231_d108 = 0 mm, d2396_d2232_d109 = -32.5 mm, d2397_d2233_d110 = 0 mm, d2398_d2234_d111 = 0 mm, d2399_d2235_d112 = 60 mm, d2400_d2236_d113 = 27.5 mm, d2401_d2237_d114 = 0 mm, d2402_d2238_d115 = 0 mm, d2403_d2239_d116 = 0 mm, d2405_susp_angle = 90 deg, d2418_d106 = 0 mm, d2419_d2415 = 0 mm, d2420_d2416 = -1 mm, d2421_d2417 = 1 mm, d2428_d2418_d106 = 0 mm, d2429_d2419_d2415 = 0 mm, d2430_d2420_d2416 = -1 mm, d2431_d2421_d2417 = 1 mm, d2432_d2422 = 0 mm
